# Autodesk Inventor assembly: Robot Chasis
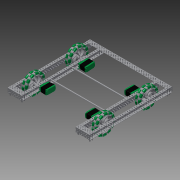
[picture p0: Inventor's stored thumbnail of the model, 180x180]
Saved by Autodesk Inventor 2015 (Build 190159000, 159)
## iProperties
Created: 2016-09-21
Part Number: Robot Chasis
Document SubType Name: Assembly
Designer: Leo
Author: Leo
## Documents named in this file (10)
- C:\Users\L\Google Drive\StarStuckProject\Starstruck\Prototypes\Robot Chasis.iam
- C:\Users\L\Google Drive\StarStuckProject\Starstruck\Imported Components\Angle 2x2x35\Angle 2x2x35.ipt
- C:\Users\L\Google Drive\StarStuckProject\Starstruck\Prototypes\Drive Inside Bracket.iam
- C:\Users\L\Google Drive\StarStuckProject\Starstruck\Prototypes\Drive Outside Bracket.iam
- C:\Users\L\Google Drive\StarStuckProject\Starstruck\Imported Components\Large Screw 1.5in\Large Screw 1.5in.ipt
- C:\Users\L\Google Drive\StarStuckProject\Starstruck\Imported Components\Lock Nut\Lock Nut.ipt
- C:\Users\L\Google Drive\StarStuckProject\Starstruck\Prototypes\Motor and Wheel.iam
- C:\Users\L\Google Drive\StarStuckProject\Starstruck\Imported Components\Angle 2x2x35\Angle 2x2x7 21 Holes Apart.ipt
- C:\Users\L\Google Drive\StarStuckProject\Starstruck\Prototypes\11.5 in Spacer.iam
- C:\Users\L\Google Drive\StarStuckProject\Starstruck\Imported Components\Large Screw .500In\Large Screw .500In.ipt
## Components (48 placed, 9 different names)
1. Angle 2x2x35:1 — Mate:9, Mate:10, Mate:11, Mate:12, Mate:13, Mate:14, Mate:15, Mate:16, Flush:5, Flush:6, Flush:7, Flush:8, Mate:17, Mate:22, Mate:23, Mate:24, Tangent:53, Tangent:54, Tangent:55, Tangent:56, Tangent:57, Tangent:58, Tangent:59, Tangent:60, Mate:60, Mate:61, Mate:62, Mate:63
2. Drive Outside Bracket:1 [sub-assembly] — Mate:12, Mate:13, Flush:5, Tangent:7, Tangent:8, Tangent:14, Tangent:15, Mate:37, Mate:38, Flush:9, Mate:53, Mate:56
3. Drive Outside Bracket:2 [sub-assembly] — Mate:9, Mate:15, Flush:8, Tangent:1, Tangent:2, Tangent:9, Tangent:10, Mate:47, Mate:50
4. Drive Inside Bracket:1 [sub-assembly] — Mate:10, Mate:16, Flush:7, Tangent:3, Tangent:4, Tangent:11, Tangent:12, Mate:41, Mate:42, Mate:43, Tangent:31, Tangent:32, Tangent:33, Tangent:34, Tangent:37, Tangent:38, Mate:46, Tangent:39, Tangent:40, Mate:48, Mate:49, Mate:51
5. Drive Inside Bracket:2 [sub-assembly] — Mate:11, Mate:14, Flush:6, Tangent:5, Tangent:6, Tangent:13, Tangent:16, Mate:39, Mate:40, Tangent:29, Tangent:30, Mate:44, Mate:45, Tangent:35, Tangent:36, Tangent:41, Tangent:42, Mate:52, Mate:54, Tangent:43, Tangent:44, Mate:55, Mate:57, Mate:58
6. Large Screw 1.5in:1 — Mate:24, Tangent:14, Tangent:15, Insert:9
7. Large Screw 1.5in:2 — Mate:23, Tangent:13, Tangent:16, Insert:8
8. Large Screw 1.5in:3 — Mate:22, Tangent:11, Tangent:12, Insert:7
9. Large Screw 1.5in:4 — Tangent:5, Tangent:6, Insert:4
10. Large Screw 1.5in:5 — Tangent:7, Tangent:8, Insert:5
11. Large Screw 1.5in:6 — Tangent:3, Tangent:4, Insert:3
12. Large Screw 1.5in:7 — Tangent:1, Tangent:2, Insert:2
13. Large Screw 1.5in:8 — Mate:17, Tangent:9, Tangent:10, Insert:6
14. Lock Nut:1 — Insert:2
15. Lock Nut:2 — Insert:4, Mate:58
16. Lock Nut:3 — Insert:5
17. Lock Nut:4 — Insert:6
18. Lock Nut:5 — Insert:7
19. Lock Nut:6 — Insert:8
20. Lock Nut:7 — Insert:9
21. Lock Nut:8 — Insert:3
22. Angle 2x2x7 21 Holes Apart:1 — Mate:37, Mate:38, Flush:9, Mate:59, Tangent:45, Tangent:46, Tangent:47, Tangent:48, Tangent:49, Tangent:50, Tangent:51, Tangent:52, Mate:64, Mate:65, Mate:66
23. 11.5 in Spacer:1 [sub-assembly] — Tangent:25, Tangent:27, Mate:44
24. 11.5 in Spacer:2 [sub-assembly] — Tangent:26, Tangent:28, Mate:40, Mate:43
25. Large Screw .500In:1 — Tangent:26, Mate:42, Tangent:31, Tangent:32
26. Large Screw .500In:2 — Tangent:27, Mate:45, Tangent:35, Tangent:36
27. Large Screw .500In:3 — Tangent:25, Mate:41, Tangent:33, Tangent:34
28. Large Screw .500In:4 — Tangent:28, Mate:39, Tangent:29, Tangent:30
29. Motor and Wheel:1 [sub-assembly] — Tangent:37, Tangent:38, Mate:46, Mate:47, Mate:51
30. Motor and Wheel:2 [sub-assembly] — Tangent:39, Tangent:40, Mate:48, Mate:49, Mate:50
31. Motor and Wheel:3 [sub-assembly] — Tangent:41, Tangent:42, Mate:52, Mate:53, Mate:54
32. Motor and Wheel:4 [sub-assembly] — Tangent:43, Tangent:44, Mate:55, Mate:56, Mate:57
33. Large Screw 1.5in:9 — Mate:59, Tangent:45, Tangent:46
34. Lock Nut:9
35. Large Screw 1.5in:10 — Tangent:51, Tangent:52, Mate:65
36. Lock Nut:10
37. Large Screw 1.5in:11 — Tangent:47, Tangent:48, Mate:64
38. Lock Nut:11
39. Large Screw 1.5in:12 — Tangent:59, Tangent:60, Mate:60
40. Lock Nut:12
41. Large Screw 1.5in:13 — Tangent:49, Tangent:50, Mate:66
42. Lock Nut:13
43. Large Screw 1.5in:14 — Tangent:55, Tangent:56, Mate:63
44. Lock Nut:14
45. Large Screw 1.5in:15 — Tangent:53, Tangent:54, Mate:62
46. Lock Nut:15
47. Large Screw 1.5in:16 — Tangent:57, Tangent:58, Mate:61
48. Lock Nut:16
## Relationships (115: Tangent 52, Mate 42, Insert 16, Flush 5)
- Mate:9: Angle 2x2x35:1 ↔ Drive Outside Bracket:2
- Mate:10: Angle 2x2x35:1 ↔ Drive Inside Bracket:1
- Mate:11: Angle 2x2x35:1 ↔ Drive Inside Bracket:2
- Mate:12: Angle 2x2x35:1 ↔ Drive Outside Bracket:1
- Mate:13: Angle 2x2x35:1 ↔ Drive Outside Bracket:1
- Mate:14: Angle 2x2x35:1 ↔ Drive Inside Bracket:2
- Mate:15: Angle 2x2x35:1 ↔ Drive Outside Bracket:2
- Mate:16: Angle 2x2x35:1 ↔ Drive Inside Bracket:1
- Flush:5: Angle 2x2x35:1 ↔ Drive Outside Bracket:1
- Flush:6: Angle 2x2x35:1 ↔ Drive Inside Bracket:2
- Flush:7: Angle 2x2x35:1 ↔ Drive Inside Bracket:1
- Flush:8: Angle 2x2x35:1 ↔ Drive Outside Bracket:2
- Mate:17: Angle 2x2x35:1 ↔ Large Screw 1.5in:8
- Mate:22: Angle 2x2x35:1 ↔ Large Screw 1.5in:3
- Mate:23: Angle 2x2x35:1 ↔ Large Screw 1.5in:2
- Mate:24: Angle 2x2x35:1 ↔ Large Screw 1.5in:1
- Tangent:1: Drive Outside Bracket:2 ↔ Large Screw 1.5in:7
- Tangent:2: Drive Outside Bracket:2 ↔ Large Screw 1.5in:7
- Tangent:3: Drive Inside Bracket:1 ↔ Large Screw 1.5in:6
- Tangent:4: Drive Inside Bracket:1 ↔ Large Screw 1.5in:6
- Tangent:5: Drive Inside Bracket:2 ↔ Large Screw 1.5in:4
- Tangent:6: Drive Inside Bracket:2 ↔ Large Screw 1.5in:4
- Tangent:7: Drive Outside Bracket:1 ↔ Large Screw 1.5in:5
- Tangent:8: Drive Outside Bracket:1 ↔ Large Screw 1.5in:5
- Tangent:9: Drive Outside Bracket:2 ↔ Large Screw 1.5in:8
- Tangent:10: Drive Outside Bracket:2 ↔ Large Screw 1.5in:8
- Tangent:11: Drive Inside Bracket:1 ↔ Large Screw 1.5in:3
- Tangent:12: Drive Inside Bracket:1 ↔ Large Screw 1.5in:3
- Tangent:13: Drive Inside Bracket:2 ↔ Large Screw 1.5in:2
- Tangent:14: Drive Outside Bracket:1 ↔ Large Screw 1.5in:1
- Tangent:15: Drive Outside Bracket:1 ↔ Large Screw 1.5in:1
- Tangent:16: Drive Inside Bracket:2 ↔ Large Screw 1.5in:2
- Insert:2 (6.5888 mm): Large Screw 1.5in:7 ↔ Lock Nut:1
- Insert:3 (6.5888 mm): Large Screw 1.5in:6 ↔ Lock Nut:8
- Insert:4 (6.5888 mm): Large Screw 1.5in:4 ↔ Lock Nut:2
- Insert:5 (6.5888 mm): Large Screw 1.5in:5 ↔ Lock Nut:3
- Insert:6 (6.5888 mm): Large Screw 1.5in:8 ↔ Lock Nut:4
- Insert:7 (6.5888 mm): Large Screw 1.5in:3 ↔ Lock Nut:5
- Insert:8 (6.5888 mm): Large Screw 1.5in:2 ↔ Lock Nut:6
- Insert:9 (6.5888 mm): Large Screw 1.5in:1 ↔ Lock Nut:7
- Mate:37: Drive Outside Bracket:1 ↔ Angle 2x2x7 21 Holes Apart:1
- Mate:38: Drive Outside Bracket:1 ↔ Angle 2x2x7 21 Holes Apart:1
- Flush:9: Drive Outside Bracket:1 ↔ Angle 2x2x7 21 Holes Apart:1
- Tangent:25: 11.5 in Spacer:1 ↔ Large Screw .500In:3
- Tangent:26: 11.5 in Spacer:2 ↔ Large Screw .500In:1
- Tangent:27: 11.5 in Spacer:1 ↔ Large Screw .500In:2
- Tangent:28: 11.5 in Spacer:2 ↔ Large Screw .500In:4
- Mate:39: Drive Inside Bracket:2 ↔ Large Screw .500In:4
- Mate:40: Drive Inside Bracket:2 ↔ 11.5 in Spacer:2
- Mate:41: Drive Inside Bracket:1 ↔ Large Screw .500In:3
- Mate:42: Drive Inside Bracket:1 ↔ Large Screw .500In:1
- Mate:43: Drive Inside Bracket:1 ↔ 11.5 in Spacer:2
- Tangent:29: Drive Inside Bracket:2 ↔ Large Screw .500In:4
- Tangent:30: Drive Inside Bracket:2 ↔ Large Screw .500In:4
- Tangent:31: Drive Inside Bracket:1 ↔ Large Screw .500In:1
- Tangent:32: Drive Inside Bracket:1 ↔ Large Screw .500In:1
- Mate:44: Drive Inside Bracket:2 ↔ 11.5 in Spacer:1
- Mate:45: Drive Inside Bracket:2 ↔ Large Screw .500In:2
- Tangent:33: Drive Inside Bracket:1 ↔ Large Screw .500In:3
- Tangent:34: Drive Inside Bracket:1 ↔ Large Screw .500In:3
- Tangent:35: Drive Inside Bracket:2 ↔ Large Screw .500In:2
- Tangent:36: Drive Inside Bracket:2 ↔ Large Screw .500In:2
- Tangent:37: Drive Inside Bracket:1 ↔ Motor and Wheel:1
- Tangent:38: Drive Inside Bracket:1 ↔ Motor and Wheel:1
- Mate:46: Drive Inside Bracket:1 ↔ Motor and Wheel:1
- Mate:47: Drive Outside Bracket:2 ↔ Motor and Wheel:1
- Tangent:39: Drive Inside Bracket:1 ↔ Motor and Wheel:2
- Tangent:40: Drive Inside Bracket:1 ↔ Motor and Wheel:2
- Mate:48: Drive Inside Bracket:1 ↔ Motor and Wheel:2
- Mate:49: Drive Inside Bracket:1 ↔ Motor and Wheel:2
- Mate:50: Drive Outside Bracket:2 ↔ Motor and Wheel:2
- Mate:51: Drive Inside Bracket:1 ↔ Motor and Wheel:1
- Tangent:41: Drive Inside Bracket:2 ↔ Motor and Wheel:3
- Tangent:42: Drive Inside Bracket:2 ↔ Motor and Wheel:3
- Mate:52: Drive Inside Bracket:2 ↔ Motor and Wheel:3
- Mate:53: Drive Outside Bracket:1 ↔ Motor and Wheel:3
- Mate:54: Drive Inside Bracket:2 ↔ Motor and Wheel:3
- Tangent:43: Drive Inside Bracket:2 ↔ Motor and Wheel:4
- Tangent:44: Drive Inside Bracket:2 ↔ Motor and Wheel:4
- Mate:55: Drive Inside Bracket:2 ↔ Motor and Wheel:4
- Mate:56: Drive Outside Bracket:1 ↔ Motor and Wheel:4
- Mate:57: Drive Inside Bracket:2 ↔ Motor and Wheel:4
- Mate:58: Drive Inside Bracket:2 ↔ Lock Nut:2
- [Insert] (6.5888 mm): Large Screw 1.5in:9 ↔ Lock Nut:9
- [Insert] (6.5888 mm): Large Screw 1.5in:10 ↔ Lock Nut:10
- [Insert] (6.5888 mm): Large Screw 1.5in:11 ↔ Lock Nut:11
- [Insert] (6.5888 mm): Large Screw 1.5in:12 ↔ Lock Nut:12
- [Insert] (6.5888 mm): Large Screw 1.5in:13 ↔ Lock Nut:13
- [Insert] (6.5888 mm): Large Screw 1.5in:14 ↔ Lock Nut:14
- [Insert] (6.5888 mm): Large Screw 1.5in:15 ↔ Lock Nut:15
- [Insert] (6.5888 mm): Large Screw 1.5in:16 ↔ Lock Nut:16
- Mate:59: Angle 2x2x7 21 Holes Apart:1 ↔ Large Screw 1.5in:9
- Tangent:45: Angle 2x2x7 21 Holes Apart:1 ↔ Large Screw 1.5in:9
- Tangent:46: Angle 2x2x7 21 Holes Apart:1 ↔ Large Screw 1.5in:9
- Tangent:47: Angle 2x2x7 21 Holes Apart:1 ↔ Large Screw 1.5in:11
- Tangent:48: Angle 2x2x7 21 Holes Apart:1 ↔ Large Screw 1.5in:11
- Tangent:49: Angle 2x2x7 21 Holes Apart:1 ↔ Large Screw 1.5in:13
- Tangent:50: Angle 2x2x7 21 Holes Apart:1 ↔ Large Screw 1.5in:13
- Tangent:51: Angle 2x2x7 21 Holes Apart:1 ↔ Large Screw 1.5in:10
- Tangent:52: Angle 2x2x7 21 Holes Apart:1 ↔ Large Screw 1.5in:10
- Tangent:53: Angle 2x2x35:1 ↔ Large Screw 1.5in:15
- Tangent:54: Angle 2x2x35:1 ↔ Large Screw 1.5in:15
- Tangent:55: Angle 2x2x35:1 ↔ Large Screw 1.5in:14
- Tangent:56: Angle 2x2x35:1 ↔ Large Screw 1.5in:14
- Tangent:57: Angle 2x2x35:1 ↔ Large Screw 1.5in:16
- Tangent:58: Angle 2x2x35:1 ↔ Large Screw 1.5in:16
- Tangent:59: Angle 2x2x35:1 ↔ Large Screw 1.5in:12
- Tangent:60: Angle 2x2x35:1 ↔ Large Screw 1.5in:12
- Mate:60: Angle 2x2x35:1 ↔ Large Screw 1.5in:12
- Mate:61: Angle 2x2x35:1 ↔ Large Screw 1.5in:16
- Mate:62: Angle 2x2x35:1 ↔ Large Screw 1.5in:15
- Mate:63: Angle 2x2x35:1 ↔ Large Screw 1.5in:14
- Mate:64: Angle 2x2x7 21 Holes Apart:1 ↔ Large Screw 1.5in:11
- Mate:65: Angle 2x2x7 21 Holes Apart:1 ↔ Large Screw 1.5in:10
- Mate:66: Angle 2x2x7 21 Holes Apart:1 ↔ Large Screw 1.5in:13
## Named parameters: d195_d121 = 6.58876 mm, d196_d121 = 6.58876 mm, d197_d121 = 6.58876 mm, d198_d121 = 6.58876 mm, d199_d121 = 6.58876 mm, d200_d121 = 6.58876 mm, d201_d121 = 6.58876 mm, d202_d121 = 6.58876 mm
